# Autodesk Inventor assembly: 217-3422-STEP
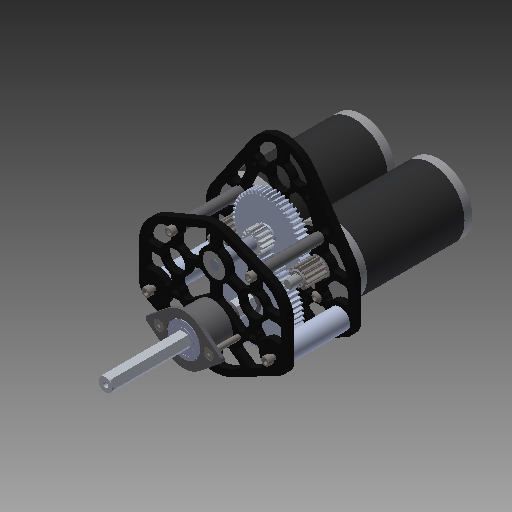
[picture p0: Inventor's stored thumbnail of the model, 512x512]
Saved by Autodesk Inventor 2018 (Build 220112000, 112)
## iProperties
Created: 2013-12-10
Part Number: 217-3422-STEP
Description: STEP AP214
Document SubType Name: Assembly
Designer: 663531
Sending System: SolidWorks 2013
Preprocessor: SwSTEP 2.0
Title: 217-3422-STEP.STEP
Revision Number: ANY
## Documents named in this file (29)
- F:\GrabCad\Resources\VEXpro Resources\Gearboxes\WCP SS Gearbox\217-3422-STEP.iam
- F:\GrabCad\Resources\VEXpro Resources\Gearboxes\WCP SS Gearbox\217-2731.ipt
- F:\GrabCad\Resources\VEXpro Resources\Gearboxes\WCP SS Gearbox\217-2733.ipt
- F:\GrabCad\Resources\VEXpro Resources\Gearboxes\WCP SS Gearbox\217-2734.ipt
- F:\GrabCad\Resources\VEXpro Resources\Gearboxes\WCP SS Gearbox\217-3099-001_12t.ipt
- F:\GrabCad\Resources\VEXpro Resources\Gearboxes\WCP SS Gearbox\217-3100-001_14t.ipt
- F:\GrabCad\Resources\VEXpro Resources\Gearboxes\WCP SS Gearbox\217-2711-002 Rev1_50t.ipt
- F:\GrabCad\Resources\VEXpro Resources\Gearboxes\WCP SS Gearbox\217-2714-002 Rev1_60t.ipt
- F:\GrabCad\Resources\VEXpro Resources\Gearboxes\WCP SS Gearbox\217-2000.ipt
- F:\GrabCad\Resources\VEXpro Resources\Gearboxes\WCP SS Gearbox\217-3421-001 Rev1.ipt
- F:\GrabCad\Resources\VEXpro Resources\Gearboxes\WCP SS Gearbox\217-3421-002 Rev1.ipt
- F:\GrabCad\Resources\VEXpro Resources\Gearboxes\WCP SS Gearbox\217-3421-004 Rev1.ipt
- F:\GrabCad\Resources\VEXpro Resources\Gearboxes\WCP SS Gearbox\217-3422-001 Rev1.ipt
- F:\GrabCad\Resources\VEXpro Resources\Gearboxes\WCP SS Gearbox\217-3422-004 Rev2.ipt
- F:\GrabCad\Resources\VEXpro Resources\Gearboxes\WCP SS Gearbox\217-3421-009 Rev1.ipt
- F:\GrabCad\Resources\VEXpro Resources\Gearboxes\WCP SS Gearbox\217-3421-010 Rev1.ipt
- F:\GrabCad\Resources\VEXpro Resources\Gearboxes\WCP SS Gearbox\217-3421-011 Rev2_97633A200.ipt
- F:\GrabCad\Resources\VEXpro Resources\Gearboxes\WCP SS Gearbox\217-3422-005 Rev1.ipt
- F:\GrabCad\Resources\VEXpro Resources\Gearboxes\WCP SS Gearbox\217-3422-006 Rev1.ipt
- F:\GrabCad\Resources\VEXpro Resources\Gearboxes\WCP SS Gearbox\217-3422-007 Rev1.ipt
- F:\GrabCad\Resources\VEXpro Resources\Gearboxes\WCP SS Gearbox\217-3422-002 Rev1.ipt
- F:\GrabCad\Resources\VEXpro Resources\Gearboxes\WCP SS Gearbox\217-3422-003 Rev1.ipt
- F:\GrabCad\Resources\VEXpro Resources\Gearboxes\WCP SS Gearbox\217-3257-001 Rev1.ipt
- F:\GrabCad\Resources\VEXpro Resources\Gearboxes\WCP SS Gearbox\217-2758-001 Rev1.ipt
- F:\GrabCad\Resources\VEXpro Resources\Gearboxes\WCP SS Gearbox\217-3259-001 Rev1.ipt
- F:\GrabCad\Resources\VEXpro Resources\Gearboxes\WCP SS Gearbox\217-3261-001 Rev1.ipt
- F:\GrabCad\Resources\VEXpro Resources\Gearboxes\WCP SS Gearbox\217-3263-001 Rev1.ipt
- F:\GrabCad\Resources\VEXpro Resources\Gearboxes\WCP SS Gearbox\217-2761-001 rev1.ipt
- F:\GrabCad\Resources\VEXpro Resources\Gearboxes\WCP SS Gearbox\217-2614-002_98430A132.ipt
## Components (43 placed, 43 different names)
1. 217-2731_1
2. 217-2733_2 — Rotational:5, Rotational:6
3. 217-2733_3 — Rotational:1, Rotational:2
4. 217-2734_4
5. 217-3099-001_12t_5
6. 217-3099-001_12t_6
7. 217-3100-001_14t_8 — Angle:1, Rotational:3, Rotational:4
8. 217-2711-002 Rev1_50t_9 — Angle:2, Rotational:4
9. 217-2714-002 Rev1_60t_10
10. 217-2000_11
11. 217-2000_13
12. 217-3421-001 Rev1_14 — Rotational:5
13. 217-3421-002 Rev1_15 — Rotational:1, Rigid:1, Rigid:2
14. 217-3421-004 Rev1_16
15. 217-3422-001 Rev1_17 — Rotational:2, Angle:1, Rotational:3, Angle:2, Rotational:6
16. 217-3422-004 Rev2_18
17. 217-3421-009 Rev1_19
18. 217-3421-009 Rev1_22
19. 217-3421-010 Rev1_23
20. 217-3421-010 Rev1_24
21. 217-3421-011 Rev2_97633A200_25
22. 217-3422-005 Rev1_26
23. 217-3422-005 Rev1_27
24. 217-3422-006 Rev1_28
25. 217-3422-006 Rev1_29
26. 217-3422-007 Rev1_30
27. 217-3422-007 Rev1_31
28. 217-3422-002 Rev1_32 — Rigid:2
29. 217-3422-002 Rev1_33 — Rigid:1
30. 217-3422-003 Rev1_34
31. 217-3422-003 Rev1_35
32. 217-3257-001 Rev1_36
33. 217-2758-001 Rev1_37
34. 217-3259-001 Rev1_38
35. 217-3261-001 Rev1_39
36. 217-3263-001 Rev1_40
37. 217-2761-001 rev1_42
38. 217-2761-001 rev1_43
39. 217-2614-002_98430A132_45
40. 217-2614-002_98430A132_46
41. 217-2614-002_98430A132_47
42. 217-2614-002_98430A132_48
43. 217-3257-001 Rev1_50
## Relationships (10: RevoluteJoint 6, Angle 2, WeldJoint 2)
- Rotational:1 [RevoluteJoint]: 217-2733_3 ↔ 217-3421-002 Rev1_15
- Rotational:2 [RevoluteJoint]: 217-2733_3 ↔ 217-3422-001 Rev1_17
- Angle:1 (0 deg): 217-3100-001_14t_8 ↔ 217-3422-001 Rev1_17
- Rotational:3 [RevoluteJoint]: 217-3100-001_14t_8 ↔ 217-3422-001 Rev1_17
- Angle:2 (0 deg): 217-2711-002 Rev1_50t_9 ↔ 217-3422-001 Rev1_17
- Rotational:4 [RevoluteJoint]: 217-3100-001_14t_8 ↔ 217-2711-002 Rev1_50t_9
- Rotational:5 [RevoluteJoint]: 217-2733_2 ↔ 217-3421-001 Rev1_14
- Rotational:6 [RevoluteJoint]: 217-2733_2 ↔ 217-3422-001 Rev1_17
- Rigid:1 [WeldJoint]: 217-3421-002 Rev1_15 ↔ 217-3422-002 Rev1_33
- Rigid:2 [WeldJoint]: 217-3421-002 Rev1_15 ↔ 217-3422-002 Rev1_32
